# Autodesk Inventor assembly: Baugruppe1
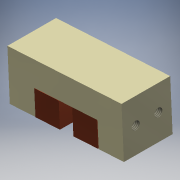
[picture p0: Inventor's stored thumbnail of the model, 180x180]
Saved by Autodesk Inventor 2018.3 (Build 223285000, 285)
## iProperties
Created: 2021-01-25
Part Number: Baugruppe1
Material: Generisch
Document SubType Name: Assembly
Designer: stege
Author: stege
## Documents named in this file (4)
- C:\Users\stege\Engineering\inventor\Baugruppe1.iam
- C:\Users\stege\Engineering\inventor\Bauteil2.ipt
- C:\Users\stege\Engineering\inventor\alublock.ipt
- C:\Users\stege\Engineering\inventor\alublock_MIR.ipt
## Components (3 placed, 3 different names)
1. Bauteil2:1 — Fluchtend:1, Fluchtend:2, Passend:1, Passend:2, Passend:3, Fluchtend:3, Passend:4
2. alublock:2 — Fluchtend:2, Passend:1, Passend:2, Fluchtend:3, Passend:4
3. alublock_MIR:1 — Fluchtend:1, Passend:3
## Relationships (7: Mate 4, Flush 3)
- Fluchtend:1 [Flush]: Bauteil2:1 ↔ alublock_MIR:1
- Fluchtend:2 [Flush]: Bauteil2:1 ↔ alublock:2
- Passend:1 [Mate]: Bauteil2:1 ↔ alublock:2
- Passend:2 [Mate] (0.25 mm): Bauteil2:1 ↔ alublock:2
- Passend:3 [Mate] (0.25 mm): Bauteil2:1 ↔ alublock_MIR:1
- Fluchtend:3 [Flush]: Bauteil2:1 ↔ alublock:2
- Passend:4 [Mate] (0.5 mm): Bauteil2:1 ↔ alublock:2
